# Autodesk Inventor assembly: CLIM_008_ClimbBox
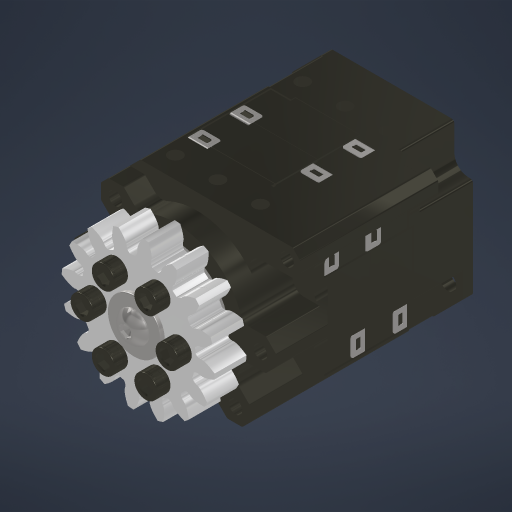
[picture p0: Inventor's stored thumbnail of the model, 512x512]
Saved by Autodesk Inventor 2024.2 (Build 282272000, 272)
## iProperties
Created: 2024-08-08
Part Number: CLIM_008_ClimbBox
Document SubType Name: Assembly
Designer: Bryan
Mass: 585.001 g
Surface Area: 1074.66 cm^2
Volume: 121.774 cm^3
Density: 4.80399 g/cm^3
Author: Bryan
## Documents named in this file (12)
- C:\Users\bobsb\OneDrive\Documents\GitHub\1622-2024-Summer-CAD-A-Thon\Climb\CLIM_008_ClimbBox.iam
- C:\Users\bobsb\OneDrive\Documents\GitHub\1622-2024-Summer-CAD-A-Thon\Climb\CLIM_006_RackGear.ipt
- C:\Users\bobsb\OneDrive\Documents\GitHub\1622-2024-Summer-CAD-A-Thon\COTS Library\Fasteners\Bolts\Button-Head\10-32\COTS_92949A265_1-2in long Stainless Steel Button Head Screw.ipt
- C:\Users\bobsb\OneDrive\Documents\GitHub\1622-2024-Summer-CAD-A-Thon\COTS Library\Fasteners\Bolts\Socket-Head\8-32\COTS_3-8in_91251A192_Black-Oxide Alloy Steel Socket Head Screw.ipt
- C:\Users\bobsb\OneDrive\Documents\GitHub\1622-2024-Summer-CAD-A-Thon\COTS Library\MAXPlanetary System\COTS_0.5inhexoutput_REV-21-2104.ipt
- C:\Users\bobsb\OneDrive\Documents\GitHub\1622-2024-Summer-CAD-A-Thon\COTS Library\MAXPlanetary System\COTS_4to1Stage_REV-21-2102.ipt
- C:\Users\bobsb\OneDrive\Documents\GitHub\1622-2024-Summer-CAD-A-Thon\COTS Library\MAXPlanetary System\COTS_5to1Stage_REV-21-2103.ipt
- C:\Users\bobsb\OneDrive\Documents\GitHub\1622-2024-Summer-CAD-A-Thon\COTS Library\MAXPlanetary System\COTS_InputStage_REV-21-2106.ipt
- C:\Users\bobsb\OneDrive\Documents\GitHub\1622-2024-Summer-CAD-A-Thon\COTS Library\MAXPlanetary System\COTS_NeoShaftAdapter_REV-21-2108.ipt
- C:\Users\bobsb\OneDrive\Documents\GitHub\1622-2024-Summer-CAD-A-Thon\Climb\CLIM_007_HexHaft.ipt
- C:\Users\bobsb\OneDrive\Documents\GitHub\1622-2024-Summer-CAD-A-Thon\COTS Library\Fasteners\Bolts\Socket-Head\10-32\COTS_91251A342_1-2in Long_Black-Oxide Alloy Steel Socket Head.ipt
- C:\Users\bobsb\OneDrive\Documents\GitHub\1622-2024-Summer-CAD-A-Thon\COTS Library\Fasteners\Washers\COTS_90107A029_316 Stainless Steel Washer.ipt
## Components (17 placed, 11 different names)
1. CLIM_006_RackGear:1 — Mate:1, Mate:2, Mate:3, Mate:4, Mate:11, Mate:12, Mate:13, Mate:14, Mate:15, Mate:16, Flush:4, Mate:30, Mate:33
2. CLIM_006_RackGear:2 — Mate:1, Mate:2, Mate:3, Mate:4, Mate:5, Mate:6, Mate:7, Mate:8, Mate:9, Mate:10, Mate:29
3. COTS_3-8in_91251A192_Black-Oxide Alloy Steel Socket Head Screw:1 — Mate:7, Mate:15
4. COTS_3-8in_91251A192_Black-Oxide Alloy Steel Socket Head Screw:2 — Mate:9, Mate:11
5. COTS_3-8in_91251A192_Black-Oxide Alloy Steel Socket Head Screw:3 — Mate:10, Mate:16
6. COTS_3-8in_91251A192_Black-Oxide Alloy Steel Socket Head Screw:4 — Mate:8, Mate:12
7. COTS_3-8in_91251A192_Black-Oxide Alloy Steel Socket Head Screw:5 — Mate:6, Mate:14
8. COTS_3-8in_91251A192_Black-Oxide Alloy Steel Socket Head Screw:6 — Mate:5, Mate:13
9. COTS_0.5inhexoutput_REV-21-2104:1 — Mate:20, Mate:21, Flush:2, Mate:25, Mate:26, Mate:27, Mate:28
10. COTS_4to1Stage_REV-21-2102:1 — Mate:18, Mate:19, Flush:1, Mate:22, Mate:23, Mate:24, Flush:3
11. COTS_5to1Stage_REV-21-2103:1 — Mate:18, Mate:19, Flush:1, Mate:20, Mate:21, Flush:2
12. COTS_InputStage_REV-21-2106:1 — Mate:17, Mate:24, Flush:3
13. COTS_NeoShaftAdapter_REV-21-2108:1 — Mate:17, Mate:22, Mate:23
14. CLIM_007_HexHaft:1 — Mate:25, Mate:26, Mate:29, Flush:4, Mate:30, Mate:34, Mate:35
15. COTS_91251A342_1-2in Long_Black-Oxide Alloy Steel Socket Head:1 — Mate:27, Mate:28
16. COTS_90107A029_316 Stainless Steel Washer:1 — Mate:33, Mate:34, Mate:36
17. COTS_92949A265_1-2in long Stainless Steel Button Head Screw:1 — Mate:35, Mate:36
## Relationships (38: Mate 34, Flush 4)
- Mate:1: CLIM_006_RackGear:1 ↔ CLIM_006_RackGear:2
- Mate:2: CLIM_006_RackGear:1 ↔ CLIM_006_RackGear:2
- Mate:3: CLIM_006_RackGear:1 ↔ CLIM_006_RackGear:2
- Mate:4: CLIM_006_RackGear:1 ↔ CLIM_006_RackGear:2
- Mate:5: CLIM_006_RackGear:2 ↔ COTS_3-8in_91251A192_Black-Oxide Alloy Steel Socket Head Screw:6
- Mate:6: CLIM_006_RackGear:2 ↔ COTS_3-8in_91251A192_Black-Oxide Alloy Steel Socket Head Screw:5
- Mate:7: CLIM_006_RackGear:2 ↔ COTS_3-8in_91251A192_Black-Oxide Alloy Steel Socket Head Screw:1
- Mate:8: CLIM_006_RackGear:2 ↔ COTS_3-8in_91251A192_Black-Oxide Alloy Steel Socket Head Screw:4
- Mate:9: CLIM_006_RackGear:2 ↔ COTS_3-8in_91251A192_Black-Oxide Alloy Steel Socket Head Screw:2
- Mate:10: CLIM_006_RackGear:2 ↔ COTS_3-8in_91251A192_Black-Oxide Alloy Steel Socket Head Screw:3
- Mate:11: CLIM_006_RackGear:1 ↔ COTS_3-8in_91251A192_Black-Oxide Alloy Steel Socket Head Screw:2
- Mate:12: CLIM_006_RackGear:1 ↔ COTS_3-8in_91251A192_Black-Oxide Alloy Steel Socket Head Screw:4
- Mate:13: CLIM_006_RackGear:1 ↔ COTS_3-8in_91251A192_Black-Oxide Alloy Steel Socket Head Screw:6
- Mate:14: CLIM_006_RackGear:1 ↔ COTS_3-8in_91251A192_Black-Oxide Alloy Steel Socket Head Screw:5
- Mate:15: CLIM_006_RackGear:1 ↔ COTS_3-8in_91251A192_Black-Oxide Alloy Steel Socket Head Screw:1
- Mate:16: CLIM_006_RackGear:1 ↔ COTS_3-8in_91251A192_Black-Oxide Alloy Steel Socket Head Screw:3
- Mate:17: COTS_InputStage_REV-21-2106:1 ↔ COTS_NeoShaftAdapter_REV-21-2108:1
- Mate:18: COTS_4to1Stage_REV-21-2102:1 ↔ COTS_5to1Stage_REV-21-2103:1
- Mate:19: COTS_4to1Stage_REV-21-2102:1 ↔ COTS_5to1Stage_REV-21-2103:1
- Flush:1: COTS_4to1Stage_REV-21-2102:1 ↔ COTS_5to1Stage_REV-21-2103:1
- Mate:20: COTS_0.5inhexoutput_REV-21-2104:1 ↔ COTS_5to1Stage_REV-21-2103:1
- Mate:21: COTS_0.5inhexoutput_REV-21-2104:1 ↔ COTS_5to1Stage_REV-21-2103:1
- Flush:2: COTS_0.5inhexoutput_REV-21-2104:1 ↔ COTS_5to1Stage_REV-21-2103:1
- Mate:22: COTS_4to1Stage_REV-21-2102:1 ↔ COTS_NeoShaftAdapter_REV-21-2108:1
- Mate:23: COTS_4to1Stage_REV-21-2102:1 ↔ COTS_NeoShaftAdapter_REV-21-2108:1
- Mate:24: COTS_4to1Stage_REV-21-2102:1 ↔ COTS_InputStage_REV-21-2106:1
- Flush:3: COTS_4to1Stage_REV-21-2102:1 ↔ COTS_InputStage_REV-21-2106:1
- Mate:25: COTS_0.5inhexoutput_REV-21-2104:1 ↔ CLIM_007_HexHaft:1
- Mate:26: COTS_0.5inhexoutput_REV-21-2104:1 ↔ CLIM_007_HexHaft:1
- Mate:27: COTS_0.5inhexoutput_REV-21-2104:1 ↔ COTS_91251A342_1-2in Long_Black-Oxide Alloy Steel Socket Head:1
- Mate:28: COTS_0.5inhexoutput_REV-21-2104:1 ↔ COTS_91251A342_1-2in Long_Black-Oxide Alloy Steel Socket Head:1
- Mate:29: CLIM_006_RackGear:2 ↔ CLIM_007_HexHaft:1
- Flush:4: CLIM_006_RackGear:1 ↔ CLIM_007_HexHaft:1
- Mate:30: CLIM_006_RackGear:1 ↔ CLIM_007_HexHaft:1
- Mate:33: CLIM_006_RackGear:1 ↔ COTS_90107A029_316 Stainless Steel Washer:1
- Mate:34: CLIM_007_HexHaft:1 ↔ COTS_90107A029_316 Stainless Steel Washer:1
- Mate:35: CLIM_007_HexHaft:1 ↔ COTS_92949A265_1-2in long Stainless Steel Button Head Screw:1
- Mate:36: COTS_90107A029_316 Stainless Steel Washer:1 ↔ COTS_92949A265_1-2in long Stainless Steel Button Head Screw:1
